# Autodesk Inventor assembly: bayonet connector
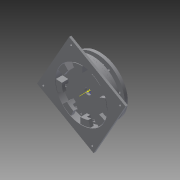
[picture p0: Inventor's stored thumbnail of the model, 180x180]
Saved by Autodesk Inventor 2015 (Build 190159000, 159)
## iProperties
Created: 2014-09-30
Part Number: bayonet connector
Document SubType Name: Assembly
Designer: ericd_000
Author: ericd_000
## Documents named in this file (5)
- C:\Users\ericd_000\Dropbox\GitHub\initial_cad\eric_cad\bayonet connector.iam
- C:\Users\ericd_000\Dropbox\GitHub\initial_cad\eric_cad\bayonet container 8.ipt
- C:\Users\ericd_000\Dropbox\GitHub\initial_cad\eric_cad\inner bayonet connector 8mk2.ipt
- C:\Users\ericd_000\Dropbox\GitHub\initial_cad\eric_cad\bay container 8 bottom.ipt
- C:\Users\ericd_000\Dropbox\GitHub\initial_cad\eric_cad\m3.ipt
## Components (5 placed, 4 different names)
1. bayonet container 8:1 — Mate:2, Mate:3, Mate:4, Mate:5, Cylindrical:1, Cylindrical:2
2. inner bayonet connector 8mk2:1 — Mate:2, Mate:3
3. bay container 8 bottom:1 — Cylindrical:3, Cylindrical:4
4. m3:1 — Mate:4, Cylindrical:1, Cylindrical:3
5. m3:2 — Mate:5, Cylindrical:2, Cylindrical:4
## Relationships (8: Mate 4, CylindricalJoint 4)
- Mate:2: bayonet container 8:1 ↔ inner bayonet connector 8mk2:1
- Mate:3: bayonet container 8:1 ↔ inner bayonet connector 8mk2:1
- Mate:4: bayonet container 8:1 ↔ m3:1
- Mate:5: bayonet container 8:1 ↔ m3:2
- Cylindrical:1: bayonet container 8:1 ↔ m3:1
- Cylindrical:2: bayonet container 8:1 ↔ m3:2
- Cylindrical:3: bay container 8 bottom:1 ↔ m3:1
- Cylindrical:4: bay container 8 bottom:1 ↔ m3:2
